# Autodesk Inventor assembly: 90 degree compact bend
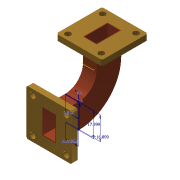
[picture p0: Inventor's stored thumbnail of the model, 180x180]
Saved by Autodesk Inventor 2015 (Build 190159000, 159)
## iProperties
Created: 2016-04-07
Part Number: 90 degree compact bend
Document SubType Name: Assembly
Designer: jad211
Author: jad211
## Documents named in this file (3)
- C:\CADFiles\EDM Machine\Detection Region\Microwave Horn Assembly\90 degree compact bend.iam
- C:\CADFiles\EDM Machine\Detection Region\Microwave Horn Assembly\curved waveguide.ipt
- C:\CADFiles\EDM Machine\Pumping Region\WG18FLANGE.ipt
## Components (3 placed, 2 different names)
1. curved waveguide:1 — Mate:1, Mate:2, Mate:3, Mate:4, Mate:5
2. WG18FLANGE:1 — Mate:1, Mate:2, Mate:3
3. WG18FLANGE:2 — Mate:4, Mate:5
## Relationships (5: Mate 5)
- Mate:1: curved waveguide:1 ↔ WG18FLANGE:1
- Mate:2: curved waveguide:1 ↔ WG18FLANGE:1
- Mate:3: curved waveguide:1 ↔ WG18FLANGE:1
- Mate:4: curved waveguide:1 ↔ WG18FLANGE:2
- Mate:5: curved waveguide:1 ↔ WG18FLANGE:2
